# Autodesk Inventor assembly: switchlockset
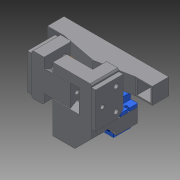
[picture p0: Inventor's stored thumbnail of the model, 180x180]
Saved by Autodesk Inventor 2015 (Build 190159000, 159)
## iProperties
Created: 2020-08-08
Part Number: switchlockset
Document SubType Name: Assembly
Designer: penta
Author: penta
## Documents named in this file (9)
- C:\Users\penta\Documents\20200806\switchlockset.iam
- C:\Users\penta\Documents\20200806\switchlock1l.ipt
- C:\Users\penta\Documents\20200806\switchlock1r.ipt
- C:\Users\penta\Documents\20200806\switchlock2l.ipt
- C:\Users\penta\Documents\20200806\switchlock2r.ipt
- C:\Users\penta\Documents\20200806\SG90 BODY.ipt
- C:\Users\penta\Documents\20200806\servolock1.ipt
- C:\Users\penta\Documents\20200806\SG90 SingleArm.ipt
- C:\Users\penta\Documents\20200806\servoarm1.ipt
## Components (8 placed, 8 different names)
1. switchlock1l:1 — 원통형:1, 강체:5, 슬라이더:1
2. switchlock1r:1 — 원통형:1, 강체:2
3. switchlock2l:1 — 강체:5
4. switchlock2r:1 — 강체:2
5. servolock1:1 — 강체:6, 슬라이더:1
6. SG90 BODY:1 — 강체:6, 회전:1
7. SG90 SingleArm:1 — 회전:1, 강체:7
8. servoarm1:1 — 강체:7
## Relationships (7: WeldJoint 4, CylindricalJoint 1, TranslationJoint 1, RevoluteJoint 1)
- 원통형:1 [CylindricalJoint]: switchlock1l:1 ↔ switchlock1r:1
- 강체:2 [WeldJoint]: switchlock1r:1 ↔ switchlock2r:1
- 강체:5 [WeldJoint]: switchlock1l:1 ↔ switchlock2l:1
- 강체:6 [WeldJoint]: servolock1:1 ↔ SG90 BODY:1
- 슬라이더:1 [TranslationJoint]: switchlock1l:1 ↔ servolock1:1
- 회전:1 [RevoluteJoint]: SG90 BODY:1 ↔ SG90 SingleArm:1
- 강체:7 [WeldJoint]: SG90 SingleArm:1 ↔ servoarm1:1
